# Autodesk Inventor assembly: 5_left_Arm
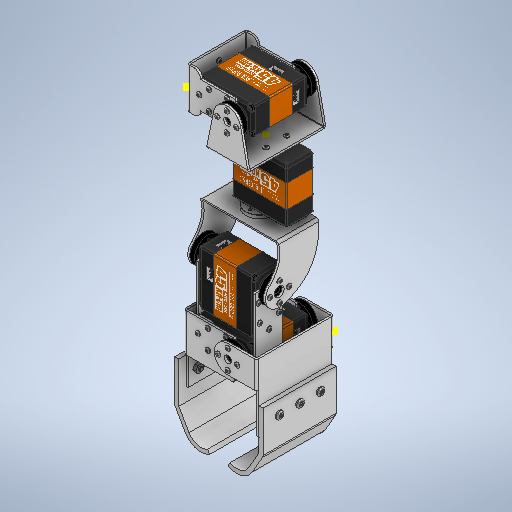
[picture p0: Inventor's stored thumbnail of the model, 512x512]
Saved by Autodesk Inventor 2026.1 (Build 301233020, 233B)
## iProperties
Created: 2025-08-13
Part Number: 5_left_Arm
Document SubType Name: Assembly
Designer: LG
Author: LG
## Documents named in this file (20)
- C:\Users\aa992\OneDrive\Desktop\RHp_Humanoid_ver1\Assembly\5_left_Arm.iam
- C:\Users\aa992\OneDrive\Desktop\RHp_Humanoid_ver1\Part\HTD-45H, Horn\HTD-45H\HTD-45H.iam
- C:\Users\aa992\OneDrive\Desktop\RHp_Humanoid_ver1\Part\HTD-45H, Horn\Horn\Top Horn.ipt
- C:\Users\aa992\OneDrive\Desktop\RHp_Humanoid_ver1\Part\Frame\Arm\axis_13_top_frame.ipt
- C:\Users\aa992\OneDrive\Desktop\RHp_Humanoid_ver1\Part\HTD-45H, Horn\Horn\Bottom Horn.ipt
- C:\Users\aa992\OneDrive\Desktop\RHp_Humanoid_ver1\Part\Frame\Arm\axis_14_bottom_frame.ipt
- C:\Users\aa992\OneDrive\Desktop\RHp_Humanoid_ver1\Part\Frame\Arm\HTD-45H_no bottom horn.ipt
- C:\Users\aa992\OneDrive\Desktop\RHp_Humanoid_ver1\Part\Frame\Arm\axis_15_bottom_frame.ipt
- C:\Users\aa992\OneDrive\Desktop\RHp_Humanoid_ver1\Part\Frame\Arm\axis_16_top_frame.ipt
- C:\Users\aa992\OneDrive\Desktop\RHp_Humanoid_ver1\Part\Frame\Arm\axis_16_bottom_frame.ipt
- C:\Users\aa992\OneDrive\Desktop\RHp_Humanoid_ver1\Part\Frame\Arm\axis_17_bottom_frame.ipt
- C:\Users\aa992\OneDrive\Desktop\RHp_Humanoid_ver1\Part\Frame\Arm\axis_17_top_frame.ipt
- C:\Users\aa992\OneDrive\Desktop\RHp_Humanoid_ver1\Part\Frame\Arm\gripper_frame.ipt
- C:\Users\aa992\OneDrive\Desktop\RHp_Humanoid_ver1\Part\Bolt, Bearing, Nut, Washer\볼트, 너트\M2x4 Bolt.ipt
- C:\Users\aa992\OneDrive\Desktop\RHp_Humanoid_ver1\Part\Bolt, Bearing, Nut, Washer\볼트, 너트\M2x6 Bolt.ipt
- C:\Users\aa992\OneDrive\Desktop\RHp_Humanoid_ver1\Part\Bolt, Bearing, Nut, Washer\볼트, 너트\M3x6 Bolt.ipt
- C:\Users\aa992\OneDrive\Desktop\RHp_Humanoid_ver1\Part\Bolt, Bearing, Nut, Washer\볼트, 너트\M3 Nut.ipt
- C:\Users\aa992\OneDrive\Desktop\RHp_Humanoid_ver1\Part\Bolt, Bearing, Nut, Washer\볼트, 너트\M3x8 Bolt.ipt
- C:\Users\aa992\OneDrive\Desktop\RHp_Humanoid_ver1\Part\HTD-45H, Horn\Horn\Top Horn silver.ipt
- C:\Users\aa992\OneDrive\Desktop\RHp_Humanoid_ver1\Part\Bolt, Bearing, Nut, Washer\M2x6 Round Bolt.ipt
## Components (104 placed, 18 different names)
1. M2x4 Bolt:80 — Rigid:146
2. M2x4 Bolt:79 — Rigid:145
3. M2x4 Bolt:78 — Rigid:144
4. M2x4 Bolt:77 — Rigid:143
5. M2x4 Bolt:76 — Rigid:139
6. M2x4 Bolt:75 — Rigid:141
7. M2x4 Bolt:74 — Rigid:138
8. M2x4 Bolt:73 — Rigid:142
9. M2x4 Bolt:72 — Rigid:140
10. M2x4 Bolt:51 — Rigid:82
11. M2x4 Bolt:54 — Rigid:84
12. M2x4 Bolt:53 — Rigid:83
13. M2x4 Bolt:52 — Rigid:85
14. Top Horn silver:1 — Rigid:147
15. axis_13_top_frame:1 — Mate:5, Mate:6, Mate:7, Rigid:82, Rigid:83, Rigid:84, Rigid:85, Rigid:138, Rigid:139, Rigid:140, Rigid:141, Rigid:142, Rigid:143, Rigid:144, Rigid:145, Rigid:146, Rigid:147
16. M2x6 Round Bolt:1 — Rigid:191
17. M2x6 Round Bolt:2 — Rigid:192
18. M2x6 Round Bolt:3 — Rigid:193
19. M2x6 Round Bolt:4 — Rigid:194
20. M2x6 Round Bolt:5 — Rigid:188
21. M2x6 Round Bolt:6 — Rigid:187
22. M2x6 Round Bolt:7 — Rigid:190
23. M2x6 Round Bolt:8 — Rigid:189
24. M2x4 Bolt:21 — Rigid:22
25. M2x4 Bolt:20 — Rigid:23
26. M2x4 Bolt:18 — Rigid:20
27. M2x4 Bolt:19 — Rigid:21
28. axis_14_bottom_frame:1 — Mate:10, Mate:11, Mate:12, Mate:13, Mate:14, Flush:4, Rigid:20, Rigid:21, Rigid:22, Rigid:23, Rigid:187, Rigid:188, Rigid:189, Rigid:190, Rigid:191, Rigid:192, Rigid:193, Rigid:194
29. Top Horn:2 — Rotational:2, Mate:10, Mate:11, Mate:12
30. Bottom Horn:1 — Mate:8, Mate:9, Flush:3
31. HTD-45H:2 [sub-assembly] — Mate:5, Mate:6, Mate:7, Rotational:2, Mate:8, Mate:9, Flush:3
32. M2x4 Bolt:25 — Rigid:24
33. M2x4 Bolt:24 — Rigid:27
34. M2x4 Bolt:23 — Rigid:26
35. M2x4 Bolt:22 — Rigid:25
36. M2x4 Bolt:30 — Rigid:32
37. M2x4 Bolt:32 — Rigid:33
38. M2x4 Bolt:31 — Rigid:34
39. M2x4 Bolt:33 — Rigid:35
40. M2x4 Bolt:26 — Rigid:28
41. M2x4 Bolt:28 — Rigid:30
42. M2x4 Bolt:27 — Rigid:29
43. M2x4 Bolt:29 — Rigid:31
44. axis_15_bottom_frame:1 — Rigid:24, Rigid:25, Rigid:26, Rigid:27, Rigid:28, Rigid:29, Rigid:30, Rigid:31, Rigid:32, Rigid:33, Rigid:34, Rigid:35, Mate:40, Mate:41, Mate:42, Mate:43, Mate:44, Flush:11
45. Top Horn silver:2 — Rotational:3, Mate:40, Mate:41, Mate:42
46. HTD-45H:3 — Mate:13, Mate:14, Flush:4, Rotational:3
47. M3x6 Bolt:1 — Rigid:179
48. M3x6 Bolt:2 — Rigid:182
49. M3x6 Bolt:3 — Rigid:180
50. M3x6 Bolt:4 — Rigid:181
51. M3 Nut:7 — Rigid:183
52. M3 Nut:8 — Rigid:186
53. M3 Nut:9 — Rigid:185
54. M3 Nut:10 — Rigid:184
55. M2x4 Bolt:55 — Rigid:93
56. M2x4 Bolt:56 — Rigid:94
57. M2x4 Bolt:57 — Rigid:92
58. M2x4 Bolt:58 — Rigid:96
59. M2x4 Bolt:59 — Rigid:95
60. M2x4 Bolt:60 — Rigid:100
61. M2x4 Bolt:61 — Rigid:97
62. M2x4 Bolt:62 — Rigid:98
63. M2x4 Bolt:63 — Rigid:99
64. axis_16_bottom_frame:1 — Mate:47, Mate:48, Flush:13, Mate:51, Flush:15, Rigid:183, Rigid:184, Rigid:185, Rigid:186
65. axis_17_bottom_frame:1 — Mate:49, Mate:50, Flush:14, Rigid:148, Rigid:159, Rigid:160, Rigid:161, Rigid:162, Rigid:163, Rigid:164, Rigid:165, Rigid:166, Rigid:176, Rigid:177, Rigid:178
66. axis_16_top_frame:1 — Rigid:86, Rigid:92, Rigid:93, Rigid:94, Rigid:95, Rigid:96, Rigid:97, Rigid:98, Rigid:99, Rigid:100, Mate:45, Mate:48, Mate:52, Rigid:179, Rigid:180, Rigid:181, Rigid:182
67. Top Horn:4 — Rotational:4, Mate:43, Mate:44, Flush:11
68. Bottom Horn:2 — Mate:29, Mate:30, Flush:6
69. HTD-45H:4 [sub-assembly] — Mate:29, Mate:30, Flush:6, Rotational:4, Rigid:86, Mate:46, Flush:12
70. M2x6 Bolt:1 — Rigid:150
71. M2x6 Bolt:2 — Rigid:152
72. M2x6 Bolt:3 — Rigid:151
73. M2x6 Bolt:4 — Rigid:153
74. M2x6 Bolt:5 — Rigid:154
75. M2x6 Bolt:6 — Rigid:155
76. M2x6 Bolt:7 — Rigid:156
77. M2x6 Bolt:8 — Rigid:157
78. M2x6 Bolt:9 — Rigid:158
79. M2x4 Bolt:81 — Rigid:160
80. M2x4 Bolt:82 — Rigid:161
81. M2x4 Bolt:83 — Rigid:159
82. M2x4 Bolt:84 — Rigid:162
83. M2x4 Bolt:85 — Rigid:164
84. M2x4 Bolt:86 — Rigid:163
85. M2x4 Bolt:87 — Rigid:165
86. M2x4 Bolt:88 — Rigid:166
87. M3x8 Bolt:1 — Rigid:170
88. M3x8 Bolt:2 — Rigid:171
89. M3x8 Bolt:3 — Rigid:172
90. M3x8 Bolt:4 — Rigid:167
91. M3x8 Bolt:5 — Rigid:168
92. M3x8 Bolt:6 — Rigid:169
93. M3 Nut:1 — Rigid:173
94. M3 Nut:2 — Rigid:175
95. M3 Nut:3 — Rigid:174
96. M3 Nut:4 — Rigid:176
97. M3 Nut:5 — Rigid:177
98. M3 Nut:6 — Rigid:178
99. axis_17_top_frame:1 — Mate:51, Flush:15, Mate:52, Rigid:149, Rigid:150, Rigid:151, Rigid:152, Rigid:153, Rigid:154, Rigid:155, Rigid:156, Rigid:157, Rigid:158, Rigid:173, Rigid:174, Rigid:175
100. gripper_frame:1 — Rigid:148, Rigid:167, Rigid:168, Rigid:169
101. gripper_frame:2 — Rigid:149, Rigid:170, Rigid:171, Rigid:172
102. Bottom Horn:3 — Mate:38, Mate:39, Flush:10
103. Top Horn:5 — Rotational:5, Mate:49, Mate:50, Flush:14
104. HTD-45H:5 [sub-assembly] — Rotational:5, Mate:38, Mate:39, Flush:10, Mate:45, Mate:46, Flush:12, Mate:47, Flush:13
## Relationships (127: WeldJoint 87, Mate 27, Flush 9, RevoluteJoint 4)
- Rotational:2 [RevoluteJoint]: Top Horn:2 ↔ HTD-45H:2
- Rotational:3 [RevoluteJoint]: Top Horn silver:2 ↔ HTD-45H:3
- Rotational:4 [RevoluteJoint]: Top Horn:4 ↔ HTD-45H:4
- Rotational:5 [RevoluteJoint]: Top Horn:5 ↔ HTD-45H:5
- Mate:5: axis_13_top_frame:1 ↔ HTD-45H:2
- Mate:6: axis_13_top_frame:1 ↔ HTD-45H:2
- Mate:7 (5 mm): axis_13_top_frame:1 ↔ HTD-45H:2
- Mate:8: Bottom Horn:1 ↔ HTD-45H:2
- Mate:9: Bottom Horn:1 ↔ HTD-45H:2
- Flush:3: Bottom Horn:1 ↔ HTD-45H:2
- Mate:10: axis_14_bottom_frame:1 ↔ Top Horn:2
- Mate:11: axis_14_bottom_frame:1 ↔ Top Horn:2
- Mate:12 (23.5 mm): axis_14_bottom_frame:1 ↔ Top Horn:2
- Mate:13: axis_14_bottom_frame:1 ↔ HTD-45H:3
- Mate:14: axis_14_bottom_frame:1 ↔ HTD-45H:3
- Flush:4: axis_14_bottom_frame:1 ↔ HTD-45H:3
- Mate:29: Bottom Horn:2 ↔ HTD-45H:4
- Mate:30: Bottom Horn:2 ↔ HTD-45H:4
- Flush:6: Bottom Horn:2 ↔ HTD-45H:4
- Mate:38: Bottom Horn:3 ↔ HTD-45H:5
- Mate:39: Bottom Horn:3 ↔ HTD-45H:5
- Flush:10: Bottom Horn:3 ↔ HTD-45H:5
- Rigid:20 [WeldJoint]: M2x4 Bolt:18 ↔ axis_14_bottom_frame:1
- Rigid:21 [WeldJoint]: M2x4 Bolt:19 ↔ axis_14_bottom_frame:1
- Rigid:22 [WeldJoint]: M2x4 Bolt:21 ↔ axis_14_bottom_frame:1
- Rigid:23 [WeldJoint]: M2x4 Bolt:20 ↔ axis_14_bottom_frame:1
- Rigid:24 [WeldJoint]: M2x4 Bolt:25 ↔ axis_15_bottom_frame:1
- Rigid:25 [WeldJoint]: M2x4 Bolt:22 ↔ axis_15_bottom_frame:1
- Rigid:26 [WeldJoint]: M2x4 Bolt:23 ↔ axis_15_bottom_frame:1
- Rigid:27 [WeldJoint]: M2x4 Bolt:24 ↔ axis_15_bottom_frame:1
- Rigid:28 [WeldJoint]: M2x4 Bolt:26 ↔ axis_15_bottom_frame:1
- Rigid:29 [WeldJoint]: M2x4 Bolt:27 ↔ axis_15_bottom_frame:1
- Rigid:30 [WeldJoint]: M2x4 Bolt:28 ↔ axis_15_bottom_frame:1
- Rigid:31 [WeldJoint]: M2x4 Bolt:29 ↔ axis_15_bottom_frame:1
- Rigid:32 [WeldJoint]: M2x4 Bolt:30 ↔ axis_15_bottom_frame:1
- Rigid:33 [WeldJoint]: M2x4 Bolt:32 ↔ axis_15_bottom_frame:1
- Rigid:34 [WeldJoint]: M2x4 Bolt:31 ↔ axis_15_bottom_frame:1
- Rigid:35 [WeldJoint]: M2x4 Bolt:33 ↔ axis_15_bottom_frame:1
- Rigid:82 [WeldJoint]: M2x4 Bolt:51 ↔ axis_13_top_frame:1
- Rigid:83 [WeldJoint]: M2x4 Bolt:53 ↔ axis_13_top_frame:1
- Rigid:84 [WeldJoint]: M2x4 Bolt:54 ↔ axis_13_top_frame:1
- Rigid:85 [WeldJoint]: M2x4 Bolt:52 ↔ axis_13_top_frame:1
- Rigid:86 [WeldJoint]: axis_16_top_frame:1 ↔ HTD-45H:4
- Rigid:92 [WeldJoint]: M2x4 Bolt:57 ↔ axis_16_top_frame:1
- Rigid:93 [WeldJoint]: M2x4 Bolt:55 ↔ axis_16_top_frame:1
- Rigid:94 [WeldJoint]: M2x4 Bolt:56 ↔ axis_16_top_frame:1
- Rigid:95 [WeldJoint]: M2x4 Bolt:59 ↔ axis_16_top_frame:1
- Rigid:96 [WeldJoint]: M2x4 Bolt:58 ↔ axis_16_top_frame:1
- Rigid:97 [WeldJoint]: M2x4 Bolt:61 ↔ axis_16_top_frame:1
- Rigid:98 [WeldJoint]: M2x4 Bolt:62 ↔ axis_16_top_frame:1
- Rigid:99 [WeldJoint]: M2x4 Bolt:63 ↔ axis_16_top_frame:1
- Rigid:100 [WeldJoint]: M2x4 Bolt:60 ↔ axis_16_top_frame:1
- Rigid:138 [WeldJoint]: M2x4 Bolt:74 ↔ axis_13_top_frame:1
- Rigid:139 [WeldJoint]: M2x4 Bolt:76 ↔ axis_13_top_frame:1
- Rigid:140 [WeldJoint]: M2x4 Bolt:72 ↔ axis_13_top_frame:1
- Rigid:141 [WeldJoint]: M2x4 Bolt:75 ↔ axis_13_top_frame:1
- Rigid:142 [WeldJoint]: M2x4 Bolt:73 ↔ axis_13_top_frame:1
- Rigid:143 [WeldJoint]: M2x4 Bolt:77 ↔ axis_13_top_frame:1
- Rigid:144 [WeldJoint]: M2x4 Bolt:78 ↔ axis_13_top_frame:1
- Rigid:145 [WeldJoint]: M2x4 Bolt:79 ↔ axis_13_top_frame:1
- Rigid:146 [WeldJoint]: M2x4 Bolt:80 ↔ axis_13_top_frame:1
- Rigid:147 [WeldJoint]: Top Horn silver:1 ↔ axis_13_top_frame:1
- Mate:40: axis_15_bottom_frame:1 ↔ Top Horn silver:2
- Mate:41: axis_15_bottom_frame:1 ↔ Top Horn silver:2
- Mate:42: axis_15_bottom_frame:1 ↔ Top Horn silver:2
- Mate:43: axis_15_bottom_frame:1 ↔ Top Horn:4
- Mate:44 (30.43 mm): axis_15_bottom_frame:1 ↔ Top Horn:4
- Flush:11 (14 mm): axis_15_bottom_frame:1 ↔ Top Horn:4
- Mate:45: axis_16_top_frame:1 ↔ HTD-45H:5
- Mate:46 (3 mm): HTD-45H:4 ↔ HTD-45H:5
- Flush:12: HTD-45H:4 ↔ HTD-45H:5
- Mate:47: axis_16_bottom_frame:1 ↔ HTD-45H:5
- Mate:48: axis_16_bottom_frame:1 ↔ axis_16_top_frame:1
- Flush:13: axis_16_bottom_frame:1 ↔ HTD-45H:5
- Mate:49: axis_17_bottom_frame:1 ↔ Top Horn:5
- Mate:50: axis_17_bottom_frame:1 ↔ Top Horn:5
- Flush:14 (19.43 mm): axis_17_bottom_frame:1 ↔ Top Horn:5
- Mate:51: axis_16_bottom_frame:1 ↔ axis_17_top_frame:1
- Flush:15: axis_16_bottom_frame:1 ↔ axis_17_top_frame:1
- Mate:52 (5 mm): axis_16_top_frame:1 ↔ axis_17_top_frame:1
- Rigid:148 [WeldJoint]: axis_17_bottom_frame:1 ↔ gripper_frame:1
- Rigid:149 [WeldJoint]: axis_17_top_frame:1 ↔ gripper_frame:2
- Rigid:150 [WeldJoint]: M2x6 Bolt:1 ↔ axis_17_top_frame:1
- Rigid:151 [WeldJoint]: M2x6 Bolt:3 ↔ axis_17_top_frame:1
- Rigid:152 [WeldJoint]: M2x6 Bolt:2 ↔ axis_17_top_frame:1
- Rigid:153 [WeldJoint]: M2x6 Bolt:4 ↔ axis_17_top_frame:1
- Rigid:154 [WeldJoint]: M2x6 Bolt:5 ↔ axis_17_top_frame:1
- Rigid:155 [WeldJoint]: M2x6 Bolt:6 ↔ axis_17_top_frame:1
- Rigid:156 [WeldJoint]: M2x6 Bolt:7 ↔ axis_17_top_frame:1
- Rigid:157 [WeldJoint]: M2x6 Bolt:8 ↔ axis_17_top_frame:1
- Rigid:158 [WeldJoint]: M2x6 Bolt:9 ↔ axis_17_top_frame:1
- Rigid:159 [WeldJoint]: axis_17_bottom_frame:1 ↔ M2x4 Bolt:83
- Rigid:160 [WeldJoint]: axis_17_bottom_frame:1 ↔ M2x4 Bolt:81
- Rigid:161 [WeldJoint]: axis_17_bottom_frame:1 ↔ M2x4 Bolt:82
- Rigid:162 [WeldJoint]: axis_17_bottom_frame:1 ↔ M2x4 Bolt:84
- Rigid:163 [WeldJoint]: axis_17_bottom_frame:1 ↔ M2x4 Bolt:86
- Rigid:164 [WeldJoint]: axis_17_bottom_frame:1 ↔ M2x4 Bolt:85
- Rigid:165 [WeldJoint]: axis_17_bottom_frame:1 ↔ M2x4 Bolt:87
- Rigid:166 [WeldJoint]: axis_17_bottom_frame:1 ↔ M2x4 Bolt:88
- Rigid:167 [WeldJoint]: M3x8 Bolt:4 ↔ gripper_frame:1
- Rigid:168 [WeldJoint]: M3x8 Bolt:5 ↔ gripper_frame:1
- Rigid:169 [WeldJoint]: M3x8 Bolt:6 ↔ gripper_frame:1
- Rigid:170 [WeldJoint]: M3x8 Bolt:1 ↔ gripper_frame:2
- Rigid:171 [WeldJoint]: M3x8 Bolt:2 ↔ gripper_frame:2
- Rigid:172 [WeldJoint]: M3x8 Bolt:3 ↔ gripper_frame:2
- Rigid:173 [WeldJoint]: M3 Nut:1 ↔ axis_17_top_frame:1
- Rigid:174 [WeldJoint]: M3 Nut:3 ↔ axis_17_top_frame:1
- Rigid:175 [WeldJoint]: M3 Nut:2 ↔ axis_17_top_frame:1
- Rigid:176 [WeldJoint]: axis_17_bottom_frame:1 ↔ M3 Nut:4
- Rigid:177 [WeldJoint]: axis_17_bottom_frame:1 ↔ M3 Nut:5
- Rigid:178 [WeldJoint]: axis_17_bottom_frame:1 ↔ M3 Nut:6
- Rigid:179 [WeldJoint]: M3x6 Bolt:1 ↔ axis_16_top_frame:1
- Rigid:180 [WeldJoint]: M3x6 Bolt:3 ↔ axis_16_top_frame:1
- Rigid:181 [WeldJoint]: M3x6 Bolt:4 ↔ axis_16_top_frame:1
- Rigid:182 [WeldJoint]: M3x6 Bolt:2 ↔ axis_16_top_frame:1
- Rigid:183 [WeldJoint]: M3 Nut:7 ↔ axis_16_bottom_frame:1
- Rigid:184 [WeldJoint]: M3 Nut:10 ↔ axis_16_bottom_frame:1
- Rigid:185 [WeldJoint]: M3 Nut:9 ↔ axis_16_bottom_frame:1
- Rigid:186 [WeldJoint]: M3 Nut:8 ↔ axis_16_bottom_frame:1
- Rigid:187 [WeldJoint]: M2x6 Round Bolt:6 ↔ axis_14_bottom_frame:1
- Rigid:188 [WeldJoint]: M2x6 Round Bolt:5 ↔ axis_14_bottom_frame:1
- Rigid:189 [WeldJoint]: M2x6 Round Bolt:8 ↔ axis_14_bottom_frame:1
- Rigid:190 [WeldJoint]: M2x6 Round Bolt:7 ↔ axis_14_bottom_frame:1
- Rigid:191 [WeldJoint]: M2x6 Round Bolt:1 ↔ axis_14_bottom_frame:1
- Rigid:192 [WeldJoint]: M2x6 Round Bolt:2 ↔ axis_14_bottom_frame:1
- Rigid:193 [WeldJoint]: M2x6 Round Bolt:3 ↔ axis_14_bottom_frame:1
- Rigid:194 [WeldJoint]: M2x6 Round Bolt:4 ↔ axis_14_bottom_frame:1
